# Autodesk Inventor assembly: 6Plaction-asm
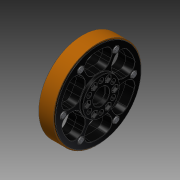
[picture p0: Inventor's stored thumbnail of the model, 180x180]
Saved by Autodesk Inventor 2014 (Build 180170000, 170)
## iProperties
Created: 2014-01-08
Part Number: 6Plaction-asm
Document SubType Name: Assembly
Designer: Kelby
Author: Unknown
Title: F:/6Plaction_asm.stp
Organization: Unknown
Description: Unknown
Sending System: Unknown
Preprocessor: XStep 1.0
Author: Kelby
## Documents named in this file (5)
- C:\Users\Kelby\Desktop\Wheels\Imported Components\6Plaction-asm\6Plaction-asm.iam
- C:\Users\Kelby\Desktop\Wheels\Imported Components\6Plaction-asm\6MW_d01.ipt
- C:\Users\Kelby\Desktop\Wheels\Imported Components\6Plaction-asm\10-32x1000shcs.ipt
- C:\Users\Kelby\Desktop\Wheels\Imported Components\6Plaction-asm\10-32_locknut.ipt
- C:\Users\Kelby\Desktop\Wheels\Imported Components\6Plaction-asm\Tread.ipt
## Components (15 placed, 4 different names)
1. 6MW_d01 — Flush:1
2. 6MW_d01:1
3. 10-32x1000shcs
4. 10-32x1000shcs:1
5. 10-32x1000shcs:2
6. 10-32x1000shcs:3
7. 10-32x1000shcs:4
8. 10-32x1000shcs:5
9. 10-32_locknut
10. 10-32_locknut:1
11. 10-32_locknut:2
12. 10-32_locknut:3
13. 10-32_locknut:4
14. 10-32_locknut:5
15. Tread:1 — Flush:1
## Relationships (1: Flush 1)
- Flush:1: 6MW_d01 ↔ Tread:1
